# Autodesk Inventor assembly: s-assy-bearing_stopper
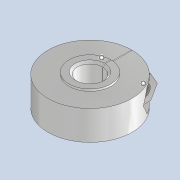
[picture p0: Inventor's stored thumbnail of the model, 180x180]
Saved by Autodesk Inventor 2022 (Build 260153000, 153)
## iProperties
Created: 2021-10-06
Part Number: s-assy-bearing_stopper
Document SubType Name: Assembly
Designer: Yuta Kage
Author: Yuta Kage
## Documents named in this file (4)
- C:\Users\yuta0\Desktop\catchrobo_shooter\s-assy-bearing_stopper.iam
- C:\Users\yuta0\Desktop\catchrobo_shooter\shooter_base7.ipt
- C:\Users\yuta0\Desktop\catchrobo_shooter\CB3-10.ipt
- C:\Users\yuta0\Desktop\catchrobo_shooter\LBNR3.ipt
## Components (3 placed, 3 different names)
1. shooter_base7:1 — メイト:1, メイト:2, メイト:4, 角度:1
2. CB3-10:1 — メイト:1, メイト:2, メイト:3
3. LBNR3:1 — メイト:3, メイト:4, 角度:1
## Relationships (5: Mate 4, Angle 1)
- メイト:1 [Mate]: shooter_base7:1 ↔ CB3-10:1
- メイト:2 [Mate]: shooter_base7:1 ↔ CB3-10:1
- メイト:3 [Mate]: CB3-10:1 ↔ LBNR3:1
- メイト:4 [Mate]: shooter_base7:1 ↔ LBNR3:1
- 角度:1 [Angle] (0 deg): shooter_base7:1 ↔ LBNR3:1
